# Autodesk Inventor assembly: Feeder
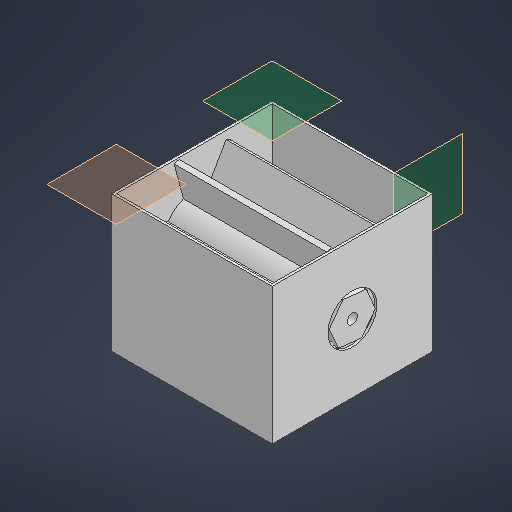
[picture p0: Inventor's stored thumbnail of the model, 512x512]
Saved by Autodesk Inventor 2026 (Build 300175050, 175E)
## iProperties
Created: 2025-11-03
Part Number: Feeder
Document SubType Name: Assembly
Designer: randy
Author: randy
## Documents named in this file (4)
- D:\CAD\DogFeeder\Feeder.iam
- D:\CAD\DogFeeder\Container.ipt
- D:\CAD\DogFeeder\Spiral.ipt
- D:\CAD\DogFeeder\Shaft.ipt
## Components (3 placed, 3 different names)
1. Container:1 — Flush:1, Flush:2, Flush:3, Mate:1, Mate:2, Mate:3
2. Spiral:1 — Mate:1, Mate:2, Mate:4
3. Shaft:1 — Mate:3, Mate:4
## Relationships (7: Mate 4, Flush 3)
- Flush:1: Container:1
- Flush:2: Container:1
- Flush:3: Container:1
- Mate:1: Container:1 ↔ Spiral:1
- Mate:2: Container:1 ↔ Spiral:1
- Mate:3: Container:1 ↔ Shaft:1
- Mate:4: Spiral:1 ↔ Shaft:1
